# Autodesk Inventor assembly: 1208
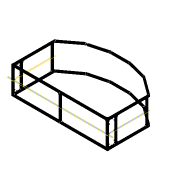
[picture p0: Inventor's stored thumbnail of the model, 180x180]
Saved by Autodesk Inventor 2020 (Build 240168000, 168)
## iProperties
Created: 2021-12-08
Part Number: 1208
Description: CAx-IF Rec.Pracs.---Model Styling and Organization---1.2---2011-12-15
Document SubType Name: Assembly
Designer: magnarecta
Sending System: 3D_Kernel_IO2017 Sp2 by CT CoreTechnologie
Preprocessor: STEP Interface 2017 Sp2 by CT CoreTechnologie
Title: 1208.stp
## Documents named in this file (48)
- D:\Documents\GitHub\Eto_Project\Hardware\Parts\MISUMI_FRAMES\model_ver4\1208.iam
- D:\Documents\GitHub\Eto_Project\Hardware\Parts\MISUMI_FRAMES\model_ver4\EFSB8-4545-2800.ipt
- D:\Documents\GitHub\Eto_Project\Hardware\Parts\MISUMI_FRAMES\model_ver4\HBKTSB8-SET(1).iam
- D:\Documents\GitHub\Eto_Project\Hardware\Parts\MISUMI_FRAMES\model_ver4\HBKTSB8-SET(2).iam
- D:\Documents\GitHub\Eto_Project\Hardware\Parts\MISUMI_FRAMES\model_ver4\EFSB8-4545-710.ipt
- D:\Documents\GitHub\Eto_Project\Hardware\Parts\MISUMI_FRAMES\model_ver4\HBKTSB8-SET(3).iam
- D:\Documents\GitHub\Eto_Project\Hardware\Parts\MISUMI_FRAMES\model_ver4\HBKTSB8-SET(4).iam
- D:\Documents\GitHub\Eto_Project\Hardware\Parts\MISUMI_FRAMES\model_ver4\HBKTSB8-SET(5).iam
- D:\Documents\GitHub\Eto_Project\Hardware\Parts\MISUMI_FRAMES\model_ver4\HBKTSB8-SET(6).iam
- D:\Documents\GitHub\Eto_Project\Hardware\Parts\MISUMI_FRAMES\model_ver4\HBKTSB8-SET(7).iam
- D:\Documents\GitHub\Eto_Project\Hardware\Parts\MISUMI_FRAMES\model_ver4\HBKTSB8-SET(8).iam
- D:\Documents\GitHub\Eto_Project\Hardware\Parts\MISUMI_FRAMES\model_ver4\HBKTSB8-SET(9).iam
- D:\Documents\GitHub\Eto_Project\Hardware\Parts\MISUMI_FRAMES\model_ver4\HBKTSB8-SET(10).iam
- D:\Documents\GitHub\Eto_Project\Hardware\Parts\MISUMI_FRAMES\model_ver4\HBKTSB8-SET(11).iam
- D:\Documents\GitHub\Eto_Project\Hardware\Parts\MISUMI_FRAMES\model_ver4\HBKTSB8-SET(12).iam
- D:\Documents\GitHub\Eto_Project\Hardware\Parts\MISUMI_FRAMES\model_ver4\HBKTSB8-SET(13).iam
- D:\Documents\GitHub\Eto_Project\Hardware\Parts\MISUMI_FRAMES\model_ver4\HBKTSB8-SET(14).iam
- D:\Documents\GitHub\Eto_Project\Hardware\Parts\MISUMI_FRAMES\model_ver4\HBKTSB8-SET(15).iam
- D:\Documents\GitHub\Eto_Project\Hardware\Parts\MISUMI_FRAMES\model_ver4\HBKTSB8-SET(16).iam
- D:\Documents\GitHub\Eto_Project\Hardware\Parts\MISUMI_FRAMES\model_ver4\HBKTSB8-SET(17).iam
- D:\Documents\GitHub\Eto_Project\Hardware\Parts\MISUMI_FRAMES\model_ver4\HBKTSB8-SET(18).iam
- D:\Documents\GitHub\Eto_Project\Hardware\Parts\MISUMI_FRAMES\model_ver4\HBKTSB8-SET(19).iam
- D:\Documents\GitHub\Eto_Project\Hardware\Parts\MISUMI_FRAMES\model_ver4\HBKTSB8-SET(20).iam
- D:\Documents\GitHub\Eto_Project\Hardware\Parts\MISUMI_FRAMES\model_ver4\HBKTSB8-SET(21).iam
- D:\Documents\GitHub\Eto_Project\Hardware\Parts\MISUMI_FRAMES\model_ver4\HBKTSB8-SET(22).iam
- D:\Documents\GitHub\Eto_Project\Hardware\Parts\MISUMI_FRAMES\model_ver4\HBKTSB8-SET(23).iam
- D:\Documents\GitHub\Eto_Project\Hardware\Parts\MISUMI_FRAMES\model_ver4\HBKTSB8-SET(24).iam
- D:\Documents\GitHub\Eto_Project\Hardware\Parts\MISUMI_FRAMES\model_ver4\HBKTSB8-SET(25).iam
- D:\Documents\GitHub\Eto_Project\Hardware\Parts\MISUMI_FRAMES\model_ver4\HBKTSB8-SET(26).iam
- D:\Documents\GitHub\Eto_Project\Hardware\Parts\MISUMI_FRAMES\model_ver4\HBKTSB8-SET(27).iam
- D:\Documents\GitHub\Eto_Project\Hardware\Parts\MISUMI_FRAMES\model_ver4\HBKTSB8-SET(28).iam
- D:\Documents\GitHub\Eto_Project\Hardware\Parts\MISUMI\EFSB8-4545-1150-RSV_Autodesk_Inventor_2020_20211208\EFSB8-4545-1150-RSV.ipt
- D:\Documents\GitHub\Eto_Project\Hardware\Parts\MISUMI\HBLTBBN45-SET_Autodesk_Inventor_2020_20211206\AIS2020\HBLTBBN45.iam
- D:\Documents\GitHub\Eto_Project\Hardware\Parts\MISUMI\EFSB8-4545-600-LSV-RSV_Autodesk_Inventor_2020_20211208\EFSB8-4545-600-LSV-RSV.ipt
- D:\Documents\GitHub\Eto_Project\Hardware\Parts\MISUMI\EFSB8-4545-500-LSV-RSV_Autodesk_Inventor_2020_20211208\EFSB8-4545-500-LSV-RSV.ipt
- D:\Documents\GitHub\Eto_Project\Hardware\Parts\MISUMI\HBLTBBN45-SET_Autodesk_Inventor_2020_20211206\AIS2020\HBLTBBN45_MIR.iam
- D:\Documents\GitHub\Eto_Project\Hardware\Parts\MISUMI\EFSB8-4545-600-LSV-RSV_Autodesk_Inventor_2020_20211208\EFSB8-4545-600-LSV-RSV_MIR.ipt
- D:\Documents\GitHub\Eto_Project\Hardware\Parts\MISUMI\EFSB8-4545-500-LSV-RSV_Autodesk_Inventor_2020_20211208\EFSB8-4545-500-LSV-RSV_MIR.ipt
- D:\Documents\GitHub\Eto_Project\Hardware\Parts\MISUMI\HBLTBBN45-SET_Autodesk_Inventor_2020_20211206\AIS2020\HBLTBBN45_MIR1.iam
- D:\Documents\GitHub\Eto_Project\Hardware\Parts\MISUMI\EFSB8-4545-600-LSV-RSV_Autodesk_Inventor_2020_20211208\EFSB8-4545-600-LSV-RSV_MIR1.ipt
- D:\Documents\GitHub\Eto_Project\Hardware\Parts\MISUMI\EFSB8-4545-500-LSV-RSV_Autodesk_Inventor_2020_20211208\EFSB8-4545-500-LSV-RSV_MIR1.ipt
- D:\Documents\GitHub\Eto_Project\Hardware\Parts\MISUMI\HBLTBBN45-SET_Autodesk_Inventor_2020_20211206\AIS2020\HBLTBBN45_MIR_MIR.iam
- D:\Documents\GitHub\Eto_Project\Hardware\Parts\MISUMI\EFSB8-4545-600-LSV-RSV_Autodesk_Inventor_2020_20211208\EFSB8-4545-600-LSV-RSV_MIR_MIR.ipt
- D:\Documents\GitHub\Eto_Project\Hardware\Parts\MISUMI\EFSB8-4545-500-LSV-RSV_Autodesk_Inventor_2020_20211208\EFSB8-4545-500-LSV-RSV_MIR_MIR.ipt
- D:\Documents\GitHub\Eto_Project\Hardware\Parts\MISUMI\HCBRB8-45_Autodesk_Inventor_2020_20211211\HCBRB8-45.ipt
- D:\Documents\GitHub\Eto_Project\Hardware\Parts\MISUMI\HCBRB8-45_Autodesk_Inventor_2020_20211211\HCBRB8-45_MIR.ipt
- D:\Documents\GitHub\Eto_Project\Hardware\Parts\MISUMI\HCBRB8-45_Autodesk_Inventor_2020_20211211\HCBRB8-45_MIR2.ipt
- D:\Documents\GitHub\Eto_Project\Hardware\Parts\MISUMI\HCBRB8-45_Autodesk_Inventor_2020_20211211\HCBRB8-45_MIR_MIR1.ipt
## Components (79 placed, 47 different names)
1. EFSB8-4545-2800 — メイト:1, フラッシュ:1, メイト:5, メイト:11, フラッシュ:26
2. HBKTSB8-SET(1) [sub-assembly]
3. EFSB8-4545-1150-RSV:1 — メイト:1, メイト:2, フラッシュ:1, メイト:9, フラッシュ:5, フラッシュ:6, フラッシュ:9
4. HBKTSB8-SET(2) [sub-assembly]
5. EFSB8-4545-710 — メイト:31, フラッシュ:46, メイト:34, メイト:38, フラッシュ:56
6. HBKTSB8-SET(3) [sub-assembly]
7. HBKTSB8-SET(4) [sub-assembly] — メイト:2
8. EFSB8-4545-710:1
9. HBKTSB8-SET(5) [sub-assembly]
10. HBKTSB8-SET(6) [sub-assembly]
11. EFSB8-4545-2800:1 — メイト:3, メイト:6
12. HBKTSB8-SET(7) [sub-assembly]
13. HBKTSB8-SET(8) [sub-assembly]
14. HBKTSB8-SET(9) [sub-assembly]
15. HBKTSB8-SET(10) [sub-assembly]
16. HBKTSB8-SET(11) [sub-assembly]
17. HBKTSB8-SET(12) [sub-assembly]
18. EFSB8-4545-710:2
19. HBKTSB8-SET(13) [sub-assembly]
20. HBKTSB8-SET(14) [sub-assembly]
21. HBKTSB8-SET(15) [sub-assembly]
22. HBKTSB8-SET(16) [sub-assembly]
23. EFSB8-4545-710:3 — フラッシュ:2, メイト:30, フラッシュ:45, メイト:35, メイト:39, フラッシュ:57
24. HBKTSB8-SET(17) [sub-assembly] — メイト:40
25. HBKTSB8-SET(18) [sub-assembly] — メイト:32, 50
26. HBKTSB8-SET(19) [sub-assembly]
27. HBKTSB8-SET(20) [sub-assembly]
28. EFSB8-4545-710:4 — フラッシュ:10
29. HBKTSB8-SET(21) [sub-assembly]
30. HBKTSB8-SET(22) [sub-assembly]
31. HBKTSB8-SET(23) [sub-assembly]
32. HBKTSB8-SET(24) [sub-assembly]
33. EFSB8-4545-710:5 — メイト:4
34. HBKTSB8-SET(25) [sub-assembly]
35. HBKTSB8-SET(26) [sub-assembly]
36. EFSB8-4545-710:6 — フラッシュ:3, フラッシュ:4, メイト:7, メイト:8
37. HBKTSB8-SET(27) [sub-assembly]
38. HBKTSB8-SET(28) [sub-assembly]
39. EFSB8-4545-1150-RSV:2 — メイト:3, フラッシュ:2, メイト:4, メイト:29, フラッシュ:44, フラッシュ:48
40. EFSB8-4545-1150-RSV:3 — メイト:6, フラッシュ:4, メイト:7
41. EFSB8-4545-1150-RSV:4 — メイト:5, フラッシュ:3, メイト:8
42. HBLTBBN45:2 [sub-assembly] — メイト:9, フラッシュ:5, フラッシュ:6, メイト:10, フラッシュ:7, フラッシュ:8
43. EFSB8-4545-600-LSV-RSV:1 — メイト:10, フラッシュ:7, フラッシュ:8, メイト:12, フラッシュ:12, フラッシュ:13
44. EFSB8-4545-500-LSV-RSV:1 — フラッシュ:9, メイト:11, フラッシュ:11, メイト:13, フラッシュ:14, フラッシュ:15
45. HBLTBBN45:3 [sub-assembly] — メイト:12, フラッシュ:12, フラッシュ:13, メイト:15, フラッシュ:16
46. HBLTBBN45:4 [sub-assembly] — メイト:13, フラッシュ:14, フラッシュ:15, メイト:14, フラッシュ:17, フラッシュ:18
47. EFSB8-4545-500-LSV-RSV:2 — メイト:14, メイト:15, フラッシュ:16, フラッシュ:17, フラッシュ:18
48. HBLTBBN45_MIR:1 [sub-assembly] — フラッシュ:19, フラッシュ:20, メイト:16
49. EFSB8-4545-600-LSV-RSV_MIR:1 — フラッシュ:19, フラッシュ:20, メイト:16, フラッシュ:21, フラッシュ:22, メイト:17
50. HBLTBBN45_MIR:2 [sub-assembly] — フラッシュ:21, フラッシュ:22, メイト:17, フラッシュ:25, メイト:18
51. HBLTBBN45_MIR:3 [sub-assembly] — フラッシュ:23, フラッシュ:24, メイト:19
52. EFSB8-4545-500-LSV-RSV_MIR:1 — フラッシュ:23, フラッシュ:24, フラッシュ:25, メイト:18, メイト:19
53. HBLTBBN45_MIR1:1 [sub-assembly] — フラッシュ:27, フラッシュ:28, メイト:20
54. EFSB8-4545-600-LSV-RSV_MIR1:1 — フラッシュ:27, フラッシュ:28, メイト:20, フラッシュ:30, フラッシュ:31, メイト:21
55. EFSB8-4545-500-LSV-RSV_MIR1:1 — フラッシュ:29, フラッシュ:32, フラッシュ:33, メイト:22
56. HBLTBBN45_MIR1:2 [sub-assembly] — フラッシュ:30, フラッシュ:31, メイト:21, フラッシュ:36, メイト:23
57. HBLTBBN45_MIR1:3 [sub-assembly] — フラッシュ:32, フラッシュ:33, メイト:22, フラッシュ:34, フラッシュ:35, メイト:24
58. EFSB8-4545-500-LSV-RSV_MIR1:2 — フラッシュ:34, フラッシュ:35, フラッシュ:36, メイト:23, メイト:24
59. HBLTBBN45_MIR_MIR:1 [sub-assembly] — メイト:25, フラッシュ:37, フラッシュ:38
60. EFSB8-4545-600-LSV-RSV_MIR_MIR:1 — メイト:25, フラッシュ:37, フラッシュ:38, メイト:26, フラッシュ:39, フラッシュ:40
61. HBLTBBN45_MIR_MIR:2 [sub-assembly] — メイト:26, フラッシュ:39, フラッシュ:40, メイト:28, フラッシュ:41
62. HBLTBBN45_MIR_MIR:3 [sub-assembly] — メイト:27, フラッシュ:42, フラッシュ:43
63. EFSB8-4545-500-LSV-RSV_MIR_MIR:1 — メイト:27, メイト:28, フラッシュ:41, フラッシュ:42, フラッシュ:43
64. HCBRB8-45:1 — メイト:30, フラッシュ:45, フラッシュ:47, 50
65. HCBRB8-45:2 — メイト:31, フラッシュ:46, フラッシュ:47, フラッシュ:51
66. HCBRB8-45:3 — メイト:29, フラッシュ:44, メイト:32
67. HCBRB8-45_MIR:1 — フラッシュ:49, メイト:39, フラッシュ:57, フラッシュ:58, メイト:40
68. HCBRB8-45_MIR:2 — フラッシュ:49, メイト:38, フラッシュ:56, フラッシュ:58
69. HCBRB8-45_MIR:3
70. HCBRB8-45:4 — メイト:35
71. HCBRB8-45:5 — メイト:34, メイト:36, フラッシュ:51
72. HCBRB8-45_MIR2:1 — フラッシュ:59
73. HCBRB8-45_MIR2:2 — フラッシュ:59, フラッシュ:62
74. HCBRB8-45_MIR2:3
75. HCBRB8-45_MIR_MIR1:1 — フラッシュ:60, フラッシュ:61
76. HCBRB8-45_MIR_MIR1:2 — フラッシュ:60, フラッシュ:61
77. HCBRB8-45_MIR_MIR1:3
78. HCBRB8-45_MIR2:4 — フラッシュ:63
79. HCBRB8-45_MIR2:5 — フラッシュ:62, メイト:41, フラッシュ:63
## Relationships (99: Flush 59, Mate 40)
- メイト:1 [Mate]: EFSB8-4545-2800 ↔ EFSB8-4545-1150-RSV:1
- メイト:2 [Mate]: EFSB8-4545-1150-RSV:1 ↔ HBKTSB8-SET(4)
- フラッシュ:1 [Flush]: EFSB8-4545-2800 ↔ EFSB8-4545-1150-RSV:1
- メイト:3 [Mate]: EFSB8-4545-2800:1 ↔ EFSB8-4545-1150-RSV:2
- フラッシュ:2 [Flush]: EFSB8-4545-710:3 ↔ EFSB8-4545-1150-RSV:2
- メイト:4 [Mate]: EFSB8-4545-710:5 ↔ EFSB8-4545-1150-RSV:2
- メイト:5 [Mate]: EFSB8-4545-2800 ↔ EFSB8-4545-1150-RSV:4
- メイト:6 [Mate]: EFSB8-4545-2800:1 ↔ EFSB8-4545-1150-RSV:3
- フラッシュ:3 [Flush]: EFSB8-4545-710:6 ↔ EFSB8-4545-1150-RSV:4
- フラッシュ:4 [Flush]: EFSB8-4545-710:6 ↔ EFSB8-4545-1150-RSV:3
- メイト:7 [Mate]: EFSB8-4545-710:6 ↔ EFSB8-4545-1150-RSV:3
- メイト:8 [Mate]: EFSB8-4545-710:6 ↔ EFSB8-4545-1150-RSV:4
- メイト:9 [Mate]: EFSB8-4545-1150-RSV:1 ↔ HBLTBBN45:2
- フラッシュ:5 [Flush]: EFSB8-4545-1150-RSV:1 ↔ HBLTBBN45:2
- フラッシュ:6 [Flush]: EFSB8-4545-1150-RSV:1 ↔ HBLTBBN45:2
- メイト:10 [Mate]: HBLTBBN45:2 ↔ EFSB8-4545-600-LSV-RSV:1
- フラッシュ:7 [Flush]: HBLTBBN45:2 ↔ EFSB8-4545-600-LSV-RSV:1
- フラッシュ:8 [Flush]: HBLTBBN45:2 ↔ EFSB8-4545-600-LSV-RSV:1
- フラッシュ:9 [Flush]: EFSB8-4545-1150-RSV:1 ↔ EFSB8-4545-500-LSV-RSV:1
- メイト:11 [Mate] (1700 mm): EFSB8-4545-2800 ↔ EFSB8-4545-500-LSV-RSV:1
- フラッシュ:10 [Flush] (-22.5 mm): EFSB8-4545-710:4
- フラッシュ:11 [Flush] (250 mm): EFSB8-4545-500-LSV-RSV:1
- メイト:12 [Mate] (-50 mm): EFSB8-4545-600-LSV-RSV:1 ↔ HBLTBBN45:3
- フラッシュ:12 [Flush]: EFSB8-4545-600-LSV-RSV:1 ↔ HBLTBBN45:3
- フラッシュ:13 [Flush]: EFSB8-4545-600-LSV-RSV:1 ↔ HBLTBBN45:3
- メイト:13 [Mate]: EFSB8-4545-500-LSV-RSV:1 ↔ HBLTBBN45:4
- フラッシュ:14 [Flush]: EFSB8-4545-500-LSV-RSV:1 ↔ HBLTBBN45:4
- フラッシュ:15 [Flush]: EFSB8-4545-500-LSV-RSV:1 ↔ HBLTBBN45:4
- メイト:14 [Mate]: HBLTBBN45:4 ↔ EFSB8-4545-500-LSV-RSV:2
- メイト:15 [Mate] (50 mm): HBLTBBN45:3 ↔ EFSB8-4545-500-LSV-RSV:2
- フラッシュ:16 [Flush]: HBLTBBN45:3 ↔ EFSB8-4545-500-LSV-RSV:2
- フラッシュ:17 [Flush]: HBLTBBN45:4 ↔ EFSB8-4545-500-LSV-RSV:2
- フラッシュ:18 [Flush]: HBLTBBN45:4 ↔ EFSB8-4545-500-LSV-RSV:2
- フラッシュ:19 [Flush]: HBLTBBN45_MIR:1 ↔ EFSB8-4545-600-LSV-RSV_MIR:1
- フラッシュ:20 [Flush]: HBLTBBN45_MIR:1 ↔ EFSB8-4545-600-LSV-RSV_MIR:1
- メイト:16 [Mate]: HBLTBBN45_MIR:1 ↔ EFSB8-4545-600-LSV-RSV_MIR:1
- フラッシュ:21 [Flush]: EFSB8-4545-600-LSV-RSV_MIR:1 ↔ HBLTBBN45_MIR:2
- フラッシュ:22 [Flush]: EFSB8-4545-600-LSV-RSV_MIR:1 ↔ HBLTBBN45_MIR:2
- メイト:17 [Mate]: EFSB8-4545-600-LSV-RSV_MIR:1 ↔ HBLTBBN45_MIR:2
- フラッシュ:23 [Flush]: HBLTBBN45_MIR:3 ↔ EFSB8-4545-500-LSV-RSV_MIR:1
- フラッシュ:24 [Flush]: HBLTBBN45_MIR:3 ↔ EFSB8-4545-500-LSV-RSV_MIR:1
- フラッシュ:25 [Flush]: HBLTBBN45_MIR:2 ↔ EFSB8-4545-500-LSV-RSV_MIR:1
- メイト:18 [Mate]: HBLTBBN45_MIR:2 ↔ EFSB8-4545-500-LSV-RSV_MIR:1
- メイト:19 [Mate]: HBLTBBN45_MIR:3 ↔ EFSB8-4545-500-LSV-RSV_MIR:1
- フラッシュ:26 [Flush] (355 mm): EFSB8-4545-2800
- フラッシュ:27 [Flush]: HBLTBBN45_MIR1:1 ↔ EFSB8-4545-600-LSV-RSV_MIR1:1
- フラッシュ:28 [Flush]: HBLTBBN45_MIR1:1 ↔ EFSB8-4545-600-LSV-RSV_MIR1:1
- メイト:20 [Mate]: HBLTBBN45_MIR1:1 ↔ EFSB8-4545-600-LSV-RSV_MIR1:1
- フラッシュ:29 [Flush] (250 mm): EFSB8-4545-500-LSV-RSV_MIR1:1
- フラッシュ:30 [Flush]: EFSB8-4545-600-LSV-RSV_MIR1:1 ↔ HBLTBBN45_MIR1:2
- フラッシュ:31 [Flush]: EFSB8-4545-600-LSV-RSV_MIR1:1 ↔ HBLTBBN45_MIR1:2
- メイト:21 [Mate]: EFSB8-4545-600-LSV-RSV_MIR1:1 ↔ HBLTBBN45_MIR1:2
- フラッシュ:32 [Flush]: EFSB8-4545-500-LSV-RSV_MIR1:1 ↔ HBLTBBN45_MIR1:3
- フラッシュ:33 [Flush]: EFSB8-4545-500-LSV-RSV_MIR1:1 ↔ HBLTBBN45_MIR1:3
- メイト:22 [Mate]: EFSB8-4545-500-LSV-RSV_MIR1:1 ↔ HBLTBBN45_MIR1:3
- フラッシュ:34 [Flush]: HBLTBBN45_MIR1:3 ↔ EFSB8-4545-500-LSV-RSV_MIR1:2
- フラッシュ:35 [Flush]: HBLTBBN45_MIR1:3 ↔ EFSB8-4545-500-LSV-RSV_MIR1:2
- フラッシュ:36 [Flush]: HBLTBBN45_MIR1:2 ↔ EFSB8-4545-500-LSV-RSV_MIR1:2
- メイト:23 [Mate]: HBLTBBN45_MIR1:2 ↔ EFSB8-4545-500-LSV-RSV_MIR1:2
- メイト:24 [Mate]: HBLTBBN45_MIR1:3 ↔ EFSB8-4545-500-LSV-RSV_MIR1:2
- メイト:25 [Mate]: HBLTBBN45_MIR_MIR:1 ↔ EFSB8-4545-600-LSV-RSV_MIR_MIR:1
- フラッシュ:37 [Flush]: HBLTBBN45_MIR_MIR:1 ↔ EFSB8-4545-600-LSV-RSV_MIR_MIR:1
- フラッシュ:38 [Flush]: HBLTBBN45_MIR_MIR:1 ↔ EFSB8-4545-600-LSV-RSV_MIR_MIR:1
- メイト:26 [Mate]: EFSB8-4545-600-LSV-RSV_MIR_MIR:1 ↔ HBLTBBN45_MIR_MIR:2
- フラッシュ:39 [Flush]: EFSB8-4545-600-LSV-RSV_MIR_MIR:1 ↔ HBLTBBN45_MIR_MIR:2
- フラッシュ:40 [Flush]: EFSB8-4545-600-LSV-RSV_MIR_MIR:1 ↔ HBLTBBN45_MIR_MIR:2
- メイト:27 [Mate]: HBLTBBN45_MIR_MIR:3 ↔ EFSB8-4545-500-LSV-RSV_MIR_MIR:1
- メイト:28 [Mate]: HBLTBBN45_MIR_MIR:2 ↔ EFSB8-4545-500-LSV-RSV_MIR_MIR:1
- フラッシュ:41 [Flush]: HBLTBBN45_MIR_MIR:2 ↔ EFSB8-4545-500-LSV-RSV_MIR_MIR:1
- フラッシュ:42 [Flush]: HBLTBBN45_MIR_MIR:3 ↔ EFSB8-4545-500-LSV-RSV_MIR_MIR:1
- フラッシュ:43 [Flush]: HBLTBBN45_MIR_MIR:3 ↔ EFSB8-4545-500-LSV-RSV_MIR_MIR:1
- メイト:29 [Mate]: EFSB8-4545-1150-RSV:2 ↔ HCBRB8-45:3
- フラッシュ:44 [Flush] (5 mm): EFSB8-4545-1150-RSV:2 ↔ HCBRB8-45:3
- メイト:30 [Mate]: EFSB8-4545-710:3 ↔ HCBRB8-45:1
- フラッシュ:45 [Flush] (5 mm): EFSB8-4545-710:3 ↔ HCBRB8-45:1
- メイト:31 [Mate]: EFSB8-4545-710 ↔ HCBRB8-45:2
- フラッシュ:46 [Flush] (5 mm): EFSB8-4545-710 ↔ HCBRB8-45:2
- メイト:32 [Mate] (41.5 mm): HBKTSB8-SET(18) ↔ HCBRB8-45:3
- フラッシュ:47 [Flush]: HCBRB8-45:1 ↔ HCBRB8-45:2
- 50 [Mate] (40 mm): HBKTSB8-SET(18) ↔ HCBRB8-45:1
- フラッシュ:48 [Flush] (355 mm): EFSB8-4545-1150-RSV:2
- フラッシュ:49 [Flush]: HCBRB8-45_MIR:1 ↔ HCBRB8-45_MIR:2
- [Flush]: HCBRB8-45:4 ↔ HCBRB8-45:5
- メイト:34 [Mate]: EFSB8-4545-710 ↔ HCBRB8-45:5
- メイト:35 [Mate]: EFSB8-4545-710:3 ↔ HCBRB8-45:4
- メイト:36 [Mate] (-7.5 mm): HCBRB8-45:5
- フラッシュ:51 [Flush]: HCBRB8-45:2 ↔ HCBRB8-45:5
- メイト:38 [Mate]: EFSB8-4545-710 ↔ HCBRB8-45_MIR:2
- フラッシュ:56 [Flush] (5 mm): EFSB8-4545-710 ↔ HCBRB8-45_MIR:2
- メイト:39 [Mate]: EFSB8-4545-710:3 ↔ HCBRB8-45_MIR:1
- フラッシュ:57 [Flush] (5 mm): EFSB8-4545-710:3 ↔ HCBRB8-45_MIR:1
- フラッシュ:58 [Flush]: HCBRB8-45_MIR:1 ↔ HCBRB8-45_MIR:2
- メイト:40 [Mate] (40 mm): HBKTSB8-SET(17) ↔ HCBRB8-45_MIR:1
- フラッシュ:59 [Flush]: HCBRB8-45_MIR2:1 ↔ HCBRB8-45_MIR2:2
- フラッシュ:60 [Flush]: HCBRB8-45_MIR_MIR1:1 ↔ HCBRB8-45_MIR_MIR1:2
- フラッシュ:61 [Flush]: HCBRB8-45_MIR_MIR1:1 ↔ HCBRB8-45_MIR_MIR1:2
- フラッシュ:62 [Flush]: HCBRB8-45_MIR2:2 ↔ HCBRB8-45_MIR2:5
- メイト:41 [Mate] (-7.5 mm): HCBRB8-45_MIR2:5
- フラッシュ:63 [Flush]: HCBRB8-45_MIR2:4 ↔ HCBRB8-45_MIR2:5
## Named parameters: d85_d80 = 0 mm
